# Autodesk Inventor assembly: capsule.final.assembly
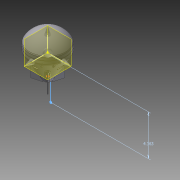
[picture p0: Inventor's stored thumbnail of the model, 180x180]
Saved by Autodesk Inventor 2011 (Build 150239000, 239)
## iProperties
Created: 2011-01-27
Part Number: capsule.final.assembly
Document SubType Name: Assembly
Designer: Casey
Author: Casey
## Documents named in this file (4)
- C:\Users\Rob\Dropbox\RockSAT-X 2011 RexSAT\capsule-launcher.design\Capsule\capsule.final.assembly.iam
- C:\Users\Rob\Dropbox\RockSAT-X 2011 RexSAT\capsule-launcher.design\Capsule\capsule.bottom.assembly.iam
- C:\Users\Rob\Dropbox\RockSAT-X 2011 RexSAT\capsule-launcher.design\Capsule\capsule.top.assembly.iam
- C:\Users\Rob\Dropbox\RockSAT-X 2011 RexSAT\capsule-launcher.design\ANSI B18.3.1M(6)\ANSI B18.3.1M - M3x0.5 x 10(1).ipt
## Components (14 placed, 3 different names)
1. capsule.bottom.assembly:1 [sub-assembly] — Mate:1, Mate:2, Mate:3
2. capsule.top.assembly:1 [sub-assembly] — Mate:1, Mate:2, Mate:3, Insert:1, Insert:2, Insert:3, Insert:4, Insert:5, Insert:6, Insert:7, Insert:8, Insert:9, Insert:10, Insert:11, Insert:12
3. Forged Socket Head Cap Screw - Metric M3x0.5 x 10:1 — Insert:1
4. Forged Socket Head Cap Screw - Metric M3x0.5 x 10:2 — Insert:2
5. Forged Socket Head Cap Screw - Metric M3x0.5 x 10:3 — Insert:3
6. Forged Socket Head Cap Screw - Metric M3x0.5 x 10:4 — Insert:4
7. Forged Socket Head Cap Screw - Metric M3x0.5 x 10:5 — Insert:5
8. Forged Socket Head Cap Screw - Metric M3x0.5 x 10:6 — Insert:6
9. Forged Socket Head Cap Screw - Metric M3x0.5 x 10:7 — Insert:7
10. Forged Socket Head Cap Screw - Metric M3x0.5 x 10:8 — Insert:8
11. Forged Socket Head Cap Screw - Metric M3x0.5 x 10:9 — Insert:9
12. Forged Socket Head Cap Screw - Metric M3x0.5 x 10:10 — Insert:10
13. Forged Socket Head Cap Screw - Metric M3x0.5 x 10:11 — Insert:11
14. Forged Socket Head Cap Screw - Metric M3x0.5 x 10:12 — Insert:12
## Relationships (15: Insert 12, Mate 3)
- Mate:1: capsule.bottom.assembly:1 ↔ capsule.top.assembly:1
- Mate:2: capsule.bottom.assembly:1 ↔ capsule.top.assembly:1
- Mate:3: capsule.bottom.assembly:1 ↔ capsule.top.assembly:1
- Insert:1: capsule.top.assembly:1 ↔ Forged Socket Head Cap Screw - Metric M3x0.5 x 10:1
- Insert:2: capsule.top.assembly:1 ↔ Forged Socket Head Cap Screw - Metric M3x0.5 x 10:2
- Insert:3: capsule.top.assembly:1 ↔ Forged Socket Head Cap Screw - Metric M3x0.5 x 10:3
- Insert:4: capsule.top.assembly:1 ↔ Forged Socket Head Cap Screw - Metric M3x0.5 x 10:4
- Insert:5: capsule.top.assembly:1 ↔ Forged Socket Head Cap Screw - Metric M3x0.5 x 10:5
- Insert:6: capsule.top.assembly:1 ↔ Forged Socket Head Cap Screw - Metric M3x0.5 x 10:6
- Insert:7: capsule.top.assembly:1 ↔ Forged Socket Head Cap Screw - Metric M3x0.5 x 10:7
- Insert:8: capsule.top.assembly:1 ↔ Forged Socket Head Cap Screw - Metric M3x0.5 x 10:8
- Insert:9: capsule.top.assembly:1 ↔ Forged Socket Head Cap Screw - Metric M3x0.5 x 10:9
- Insert:10: capsule.top.assembly:1 ↔ Forged Socket Head Cap Screw - Metric M3x0.5 x 10:10
- Insert:11: capsule.top.assembly:1 ↔ Forged Socket Head Cap Screw - Metric M3x0.5 x 10:11
- Insert:12: capsule.top.assembly:1 ↔ Forged Socket Head Cap Screw - Metric M3x0.5 x 10:12
